# Autodesk Inventor assembly: Chain Link Extractor Assembly
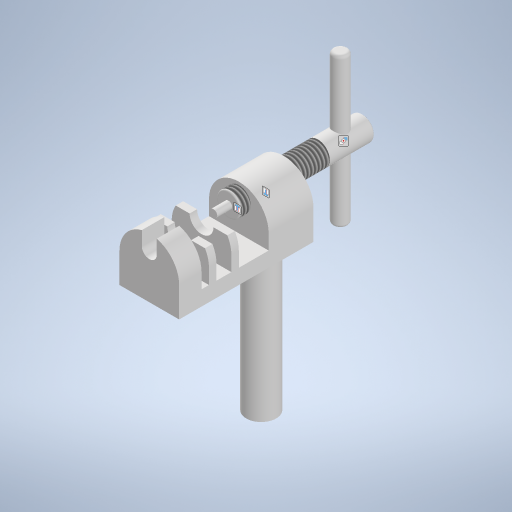
[picture p0: Inventor's stored thumbnail of the model, 512x512]
Saved by Autodesk Inventor 2023 (Build 270158030, 158C)
## iProperties
Created: 2022-11-22
Part Number: Chain Link Extractor Assembly
Document SubType Name: Assembly
Designer: Imogen Heard
Author: Imogen Heard
## Documents named in this file (6)
- C:\Users\dheard\Documents\Inventor\Inventor_Projects\Heriot Watt\Engineering Graphics\Chain Link Extractor\Chain Link Extractor Assembly.iam
- C:\Users\dheard\Documents\Inventor\Inventor_Projects\Heriot Watt\Engineering Graphics\Chain Link Extractor\Replaceable Drive Pin.ipt
- C:\Users\dheard\Documents\Inventor\Inventor_Projects\Heriot Watt\Engineering Graphics\Chain Link Extractor\Extractor Body.ipt
- C:\Users\dheard\Documents\Inventor\Inventor_Projects\Heriot Watt\Engineering Graphics\Chain Link Extractor\Drivescrew.ipt
- C:\Users\dheard\Documents\Inventor\Inventor_Projects\Heriot Watt\Engineering Graphics\Chain Link Extractor\Drivescrew Handle.ipt
- C:\Users\dheard\Documents\Inventor\Inventor_Projects\Heriot Watt\Engineering Graphics\Chain Link Extractor\Body Handle.ipt
## Components (5 placed, 5 different names)
1. Replaceable Drive Pin:1 — Insert:1
2. Extractor Body:1 — Insert:2, Insert:3
3. Drivescrew:1 — Insert:1, Mate:1, Insert:2
4. Drivescrew Handle:1 — Mate:1
5. Body Handle:1 — Insert:3
## Relationships (4: Insert 3, Mate 1)
- Insert:1 (-10 mm): Replaceable Drive Pin:1 ↔ Drivescrew:1
- Mate:1: Drivescrew:1 ↔ Drivescrew Handle:1
- Insert:2 (-18 mm): Extractor Body:1 ↔ Drivescrew:1
- Insert:3 (-10 mm): Extractor Body:1 ↔ Body Handle:1
